# Autodesk Inventor assembly: SmallSpoolAssembly
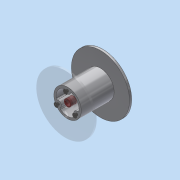
[picture p0: Inventor's stored thumbnail of the model, 180x180]
Saved by Autodesk Inventor 2017 (Build 210142000, 142)
## iProperties
Created: 2018-04-03
Part Number: SmallSpoolAssembly
Document SubType Name: Assembly
Designer: Derek Wider
Author: Derek Wider
## Documents named in this file (8)
- G:\Projects\Submarine\Submarine-project\CAD\midships\SpoolSection\SmallSpoolAssembly.iam
- G:\Projects\Submarine\Submarine-project\CAD\midships\SpoolSection\SmallSpoolEndAft.ipt
- G:\Projects\Submarine\Submarine-project\CAD\midships\SpoolSection\SmallSpoolEndFore.ipt
- G:\Projects\Submarine\Submarine-project\CAD\midships\SpoolSection\SpoolSmall.ipt
- G:\Projects\Submarine\Submarine-project\CAD\common\screws\flatPlasticScrewSmall.ipt
- G:\Projects\Submarine\Submarine-project\CAD\common\SleeveBearing.25inch.ipt
- G:\Projects\Submarine\Submarine-project\CAD\midships\SpoolSection\SpurGearLarge.ipt
- G:\Projects\Submarine\Submarine-project\CAD\common\screws\ScrewPlastic_4_20_.5inch.ipt
## Components (15 placed, 7 different names)
1. SmallSpoolEndAft:1 — Mate:1, Mate:2, Mate:3, Mate:5, Flush:1, Mate:9, Mate:10, Mate:13, Mate:14, Mate:15
2. SmallSpoolEndFore:1 — Mate:4, Mate:5, Mate:6, Flush:2, Mate:11, Mate:12
3. SpoolSmall:1 — Mate:1, Mate:2, Mate:3, Mate:4, Mate:6, Mate:7, Mate:8
4. SleeveBearing.25inch:1 — Mate:9, Mate:10
5. SleeveBearing.25inch:2 — Mate:11, Mate:12
6. SpurGearLarge:1 — Mate:13, Mate:14, Mate:15, Mate:16, Mate:17
7. flatPlasticScrewSmall:1 — Mate:7, Flush:1
8. flatPlasticScrewSmall:2
9. flatPlasticScrewSmall:3
10. flatPlasticScrewSmall:4 — Mate:8, Flush:2
11. flatPlasticScrewSmall:5
12. flatPlasticScrewSmall:6
13. ScrewPlastic_4_20_.5inch:1 — Mate:16, Mate:17
14. ScrewPlastic_4_20_.5inch:2
15. ScrewPlastic_4_20_.5inch:3
## Component patterns: (3 elements, first: flatPlasticScrewSmall:1), (3 elements, first: flatPlasticScrewSmall:4), (3 elements, first: ScrewPlastic_4_20_.5inch:1)
## Relationships (19: Mate 17, Flush 2)
- Mate:1: SmallSpoolEndAft:1 ↔ SpoolSmall:1
- Mate:2: SmallSpoolEndAft:1 ↔ SpoolSmall:1
- Mate:3: SmallSpoolEndAft:1 ↔ SpoolSmall:1
- Mate:4: SmallSpoolEndFore:1 ↔ SpoolSmall:1
- Mate:5: SmallSpoolEndAft:1 ↔ SmallSpoolEndFore:1
- Mate:6: SmallSpoolEndFore:1 ↔ SpoolSmall:1
- Mate:7: SpoolSmall:1 ↔ flatPlasticScrewSmall:1
- Flush:1: SmallSpoolEndAft:1 ↔ flatPlasticScrewSmall:1
- Mate:8: SpoolSmall:1 ↔ flatPlasticScrewSmall:4
- Flush:2: SmallSpoolEndFore:1 ↔ flatPlasticScrewSmall:4
- Mate:9: SmallSpoolEndAft:1 ↔ SleeveBearing.25inch:1
- Mate:10: SmallSpoolEndAft:1 ↔ SleeveBearing.25inch:1
- Mate:11: SmallSpoolEndFore:1 ↔ SleeveBearing.25inch:2
- Mate:12: SmallSpoolEndFore:1 ↔ SleeveBearing.25inch:2
- Mate:13: SmallSpoolEndAft:1 ↔ SpurGearLarge:1
- Mate:14: SmallSpoolEndAft:1 ↔ SpurGearLarge:1
- Mate:15: SmallSpoolEndAft:1 ↔ SpurGearLarge:1
- Mate:16: SpurGearLarge:1 ↔ ScrewPlastic_4_20_.5inch:1
- Mate:17: SpurGearLarge:1 ↔ ScrewPlastic_4_20_.5inch:1
